# Autodesk Inventor assembly: Assembly1
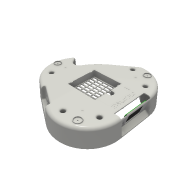
[picture p0: Inventor's stored thumbnail of the model, 180x180]
Saved by Autodesk Inventor 2016 (Build 200138000, 138)
## iProperties
Created: 2018-02-06
Part Number: Assembly1
Document SubType Name: Assembly
Designer: Juny
Author: Juny
## Documents named in this file (3)
- C:\Users\Juny\Desktop\Ateam\1612 3D 도면\bottom cover assy\Assembly1.iam
- C:\Users\Juny\Desktop\Ateam\1612 3D 도면\bottom cover assy\bottom_cover angle.ipt
- C:\Users\Juny\Desktop\Ateam\1612 3D 도면\bottom cover assy\VER.2 LCD.ipt
## Components (2 placed, 2 different names)
1. bottom_cover angle:1 — Mate:1, Angle:1
2. VER.2 LCD:1 — Mate:1, Angle:1
## Relationships (2: Mate 1, Angle 1)
- Mate:1: bottom_cover angle:1 ↔ VER.2 LCD:1
- Angle:1 (0 deg): bottom_cover angle:1 ↔ VER.2 LCD:1
